# Autodesk Inventor assembly: Robot
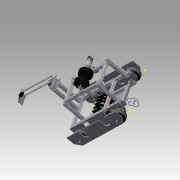
[picture p0: Inventor's stored thumbnail of the model, 180x180]
Saved by Autodesk Inventor 2016 (Build 200138000, 138)
## iProperties
Created: 2016-10-08
Part Number: Robot
Document SubType Name: Assembly
Designer: RoboticsUser
Author: RoboticsUser
## Documents named in this file (20)
- C:\Robotics\CAD\2016-17_CAD\Robot.iam
- C:\Robotics\CAD\2016-17_CAD\WheelAssemblyWFrame.iam
- C:\Robotics\CAD\COTSParts\Bosch Extrusion\Bosch 20x20 9 in.ipt
- C:\Robotics\CAD\COTSParts\Bosch Extrusion\Gusset 20x20 w screws.ipt
- C:\Robotics\CAD\COTSParts\Bosch Extrusion\Bosch 20x20 9 in - Copy.ipt
- C:\Robotics\CAD\COTSParts\Bosch Extrusion\Rexroth-6mmT-Nutm4.ipt
- C:\Robotics\CAD\COTSParts\Bosch Extrusion\Rexroth-GussetwFastenersm4x8.ipt
- C:\Robotics\CAD\COTSParts\Bosch Extrusion\Bosch 20x20 7in.ipt
- C:\Robotics\CAD\COTSParts\Bosch Extrusion\Bosch 20x20 9 in actual.ipt
- C:\Robotics\CAD\2016-17_CAD\ParticleLauncher2.0.iam
- C:\Robotics\CAD\2016-17_CAD\BBP.iam
- C:\Robotics\CAD\2016-17_CAD\ElectronicsPlate2.ipt
- C:\Robotics\CAD\COTSParts\ModernRobotics\MRI45-2204_Servo_Controller.ipt
- C:\Robotics\CAD\COTSParts\ModernRobotics\MRI45-2200_Power_Distribution_Module.ipt
- C:\Robotics\CAD\COTSParts\ModernRobotics\MRI45-2203_Motor_Controller.ipt
- C:\Robotics\CAD\COTSParts\ModernRobotics\MRI45-2201_Device_Interface.ipt
- C:\Robotics\CAD\COTSParts\Actobotics\545 parts\545400.ipt
- C:\Robotics\CAD\2016-17_CAD\PVCpipe.ipt
- C:\Robotics\CAD\COTSParts\Actobotics\545 parts\545548.ipt
- C:\Robotics\CAD\COTSParts\Actobotics\615 parts\615106.ipt
## Components (61 placed, 19 different names)
1. WheelAssemblyWFrame:1 [sub-assembly] — Mate:1, Insert:4, Insert:5, Insert:6, Flush:29, Mate:55, Flush:37, Flush:42, Mate:81, Flush:48, Flush:49, Mate:82, Flush:50, Mate:85, Flush:54, Flush:55, Mate:86
2. WheelAssemblyWFrame:2 [sub-assembly] — Mate:8, Mate:9, Flush:7, Flush:8, Insert:1, Insert:2, Insert:3, Flush:30, Flush:35, Mate:57, Mate:58, Mate:77, Mate:78, Mate:79, Flush:45, Flush:46, Flush:47, Mate:84, Flush:53, Flush:56, Mate:88, Mate:107
3. Bosch 20x20 9 in:1 — Flush:37, Mate:56, Mate:58, Mate:69, Flush:40, Mate:70, Mate:71, Mate:72, Flush:42, Mate:73, Flush:43, Mate:75, Flush:44, Mate:77
4. Gusset 20x20 w screws:1 — Mate:9, Flush:7, Mate:10, Mate:110
5. Gusset 20x20 w screws:2 — Mate:1
6. Gusset 20x20 w screws:3 — Mate:8
7. Gusset 20x20 w screws:4 — Mate:11, Flush:9
8. Bosch 20x20 9 in:2 — Mate:10, Flush:8, Mate:11, Flush:9, Flush:35, Mate:55
9. Bosch 20x20 9 in - Copy:1 — Mate:33, Flush:25, Flush:28, Flush:30, Flush:31, Mate:44, Flush:34, Mate:52, Mate:53, Mate:108, Mate:131, Mate:132, Mate:133, Mate:134, Mate:135, Flush:76
10. Rexroth-6mmT-Nutm4:1 — Insert:1
11. Rexroth-6mmT-Nutm4:2 — Insert:3, Mate:33, Flush:25
12. Rexroth-6mmT-Nutm4:3 — Insert:2
13. Bosch 20x20 9 in - Copy:2 — Mate:15, Flush:11, Mate:35, Mate:39, Flush:27, Flush:29, Flush:32, Mate:48, Flush:33, Mate:54, Mate:136, Mate:137, Mate:138, Mate:139, Flush:77
14. Rexroth-6mmT-Nutm4:4 — Insert:4
15. Rexroth-6mmT-Nutm4:5 — Insert:5
16. Rexroth-6mmT-Nutm4:6 — Insert:6, Mate:15, Flush:11
17. Bosch 20x20 9 in:3 — Flush:27, Flush:31, Mate:50, Mate:51, Mate:53, Mate:54, Flush:69
18. Bosch 20x20 9 in:4 — Mate:39, Flush:28, Flush:32, Mate:45, Mate:46, Mate:47, Mate:49, Flush:33, Flush:34, Mate:106, Mate:130
19. Gusset 20x20 w screws:5 — Mate:51, Mate:52
20. Gusset 20x20 w screws:6 — Mate:35, Mate:50
21. Gusset 20x20 w screws:7 — Mate:47, Mate:48, Mate:49
22. Gusset 20x20 w screws:8 — Mate:44, Mate:45, Mate:46
23. Rexroth-GussetwFastenersm4x8:4 — Mate:56, Mate:57
24. Gusset 20x20 w screws:11 — Mate:70, Mate:71, Mate:76
25. Gusset 20x20 w screws:12 — Mate:69, Flush:40, Mate:72, Mate:74
26. Bosch 20x20 9 in actual:1 — Mate:73, Flush:43, Mate:74, Flush:66, Mate:104, Flush:68
27. Bosch 20x20 9 in actual:2 — Mate:75, Flush:44, Mate:76, Mate:100, Mate:101, Mate:102, Flush:67, Mate:126
28. Bosch 20x20 7in:3 — Mate:79, Flush:45, Mate:80, Flush:58, Mate:91, Flush:59, Mate:94, Flush:63
29. Bosch 20x20 7in:4 — Mate:82, Mate:83, Flush:50, Mate:93, Flush:62
30. Gusset 20x20 w screws:13 — Mate:81, Flush:48, Flush:49, Mate:83
31. Gusset 20x20 w screws:14 — Mate:78, Mate:80, Flush:46, Flush:47
32. Bosch 20x20 7in:5 — Mate:84, Flush:53, Mate:89, Flush:60, Mate:98
33. Bosch 20x20 7in:6 — Mate:85, Flush:54, Mate:87, Flush:61, Mate:96, Flush:64
34. Gusset 20x20 w screws:15 — Flush:56, Mate:88, Mate:89
35. Gusset 20x20 w screws:16 — Flush:55, Mate:86, Mate:87
36. ParticleLauncher2.0:1 [sub-assembly] — Flush:58, Mate:91, Flush:59, Flush:60, Flush:61, Mate:92, Mate:95, Mate:97, Mate:99, Flush:65
37. Gusset 20x20 w screws:17 — Mate:94, Mate:95, Flush:63
38. Gusset 20x20 w screws:18 — Mate:92, Mate:93, Flush:62
39. Gusset 20x20 w screws:19 — Mate:96, Mate:97, Flush:64
40. Gusset 20x20 w screws:20 — Mate:98, Mate:99, Flush:65
41. BBP:1 [sub-assembly] — Mate:100, Mate:101, Flush:66, Mate:103, Mate:105, Mate:126
42. Gusset 20x20 w screws:21 — Mate:104, Mate:105, Flush:68
43. Gusset 20x20 w screws:22 — Mate:102, Mate:103, Flush:67
44. ElectronicsPlate2:1 — Mate:106, Flush:69, Mate:107, Mate:109, Mate:111, Mate:114, Mate:116, Mate:120, Mate:127, Mate:129
45. MRI45-2204_Servo_Controller:1 — Mate:120, Flush:73
46. MRI45-2200_Power_Distribution_Module:1 — Mate:108, Mate:109, Mate:110, Mate:112, Flush:70
47. MRI45-2203_Motor_Controller:1 — Mate:127, Flush:73, Mate:128, Flush:74
48. MRI45-2203_Motor_Controller:2 — Mate:114, Mate:115, Flush:71, Mate:117, Flush:72
49. MRI45-2203_Motor_Controller:3 — Mate:116, Mate:117, Flush:72, Mate:128, Flush:74
50. MRI45-2203_Motor_Controller:4 — Mate:111, Mate:112, Flush:70, Mate:115, Flush:71
51. MRI45-2201_Device_Interface:1 — Mate:129, Mate:130, Mate:131
52. 545400:1 — Insert:7, Insert:8
53. 545400:2 — Insert:9, Insert:10, Insert:14
54. Rexroth-6mmT-Nutm4:7 — Mate:132, Mate:133, Insert:7
55. Rexroth-6mmT-Nutm4:8 — Mate:134, Mate:135, Flush:76, Insert:8
56. Rexroth-6mmT-Nutm4:9 — Mate:136, Mate:137, Insert:10
57. Rexroth-6mmT-Nutm4:10 — Mate:138, Mate:139, Flush:77, Insert:9
58. PVCpipe:1 — Insert:12, Insert:13
59. 545548:1 — Insert:12, Insert:15
60. 545548:3 — Insert:13, Insert:14
61. 615106:1 — Insert:15
## Relationships (148: Mate 86, Flush 48, Insert 14)
- Mate:1: WheelAssemblyWFrame:1 ↔ Gusset 20x20 w screws:2
- Mate:8: WheelAssemblyWFrame:2 ↔ Gusset 20x20 w screws:3
- Mate:9: WheelAssemblyWFrame:2 ↔ Gusset 20x20 w screws:1
- Flush:7: WheelAssemblyWFrame:2 ↔ Gusset 20x20 w screws:1
- Mate:10: Gusset 20x20 w screws:1 ↔ Bosch 20x20 9 in:2
- Flush:8: WheelAssemblyWFrame:2 ↔ Bosch 20x20 9 in:2
- Mate:11: Gusset 20x20 w screws:4 ↔ Bosch 20x20 9 in:2
- Flush:9: Gusset 20x20 w screws:4 ↔ Bosch 20x20 9 in:2
- Insert:1: WheelAssemblyWFrame:2 ↔ Rexroth-6mmT-Nutm4:1
- Insert:2: WheelAssemblyWFrame:2 ↔ Rexroth-6mmT-Nutm4:3
- Insert:3: WheelAssemblyWFrame:2 ↔ Rexroth-6mmT-Nutm4:2
- Insert:4: WheelAssemblyWFrame:1 ↔ Rexroth-6mmT-Nutm4:4
- Insert:5: WheelAssemblyWFrame:1 ↔ Rexroth-6mmT-Nutm4:5
- Insert:6: WheelAssemblyWFrame:1 ↔ Rexroth-6mmT-Nutm4:6
- Mate:15: Bosch 20x20 9 in - Copy:2 ↔ Rexroth-6mmT-Nutm4:6
- Flush:11 (64.77 mm): Bosch 20x20 9 in - Copy:2 ↔ Rexroth-6mmT-Nutm4:6
- Mate:33: Bosch 20x20 9 in - Copy:1 ↔ Rexroth-6mmT-Nutm4:2
- Flush:25 (64.77 mm): Bosch 20x20 9 in - Copy:1 ↔ Rexroth-6mmT-Nutm4:2
- Mate:35: Bosch 20x20 9 in - Copy:2 ↔ Gusset 20x20 w screws:6
- Mate:39: Bosch 20x20 9 in - Copy:2 ↔ Bosch 20x20 9 in:4
- Flush:27: Bosch 20x20 9 in - Copy:2 ↔ Bosch 20x20 9 in:3
- Flush:28: Bosch 20x20 9 in - Copy:1 ↔ Bosch 20x20 9 in:4
- Flush:29 (1.6256 mm): WheelAssemblyWFrame:1 ↔ Bosch 20x20 9 in - Copy:2
- Flush:30 (1.6256 mm): WheelAssemblyWFrame:2 ↔ Bosch 20x20 9 in - Copy:1
- Flush:31 (56.896 mm): Bosch 20x20 9 in - Copy:1 ↔ Bosch 20x20 9 in:3
- Flush:32: Bosch 20x20 9 in - Copy:2 ↔ Bosch 20x20 9 in:4
- Mate:44: Bosch 20x20 9 in - Copy:1 ↔ Gusset 20x20 w screws:8
- Mate:45: Bosch 20x20 9 in:4 ↔ Gusset 20x20 w screws:8
- Mate:46: Bosch 20x20 9 in:4 ↔ Gusset 20x20 w screws:8
- Mate:47: Bosch 20x20 9 in:4 ↔ Gusset 20x20 w screws:7
- Mate:48: Bosch 20x20 9 in - Copy:2 ↔ Gusset 20x20 w screws:7
- Mate:49: Bosch 20x20 9 in:4 ↔ Gusset 20x20 w screws:7
- Flush:33: Bosch 20x20 9 in - Copy:2 ↔ Bosch 20x20 9 in:4
- Flush:34: Bosch 20x20 9 in - Copy:1 ↔ Bosch 20x20 9 in:4
- Mate:50: Bosch 20x20 9 in:3 ↔ Gusset 20x20 w screws:6
- Mate:51: Bosch 20x20 9 in:3 ↔ Gusset 20x20 w screws:5
- Mate:52: Bosch 20x20 9 in - Copy:1 ↔ Gusset 20x20 w screws:5
- Mate:53: Bosch 20x20 9 in - Copy:1 ↔ Bosch 20x20 9 in:3
- Mate:54: Bosch 20x20 9 in - Copy:2 ↔ Bosch 20x20 9 in:3
- Flush:35 (127 mm): WheelAssemblyWFrame:2 ↔ Bosch 20x20 9 in:2
- Mate:55: WheelAssemblyWFrame:1 ↔ Bosch 20x20 9 in:2
- Flush:37: WheelAssemblyWFrame:1 ↔ Bosch 20x20 9 in:1
- Mate:56: Bosch 20x20 9 in:1 ↔ Rexroth-GussetwFastenersm4x8:4
- Mate:57: WheelAssemblyWFrame:2 ↔ Rexroth-GussetwFastenersm4x8:4
- Mate:58: WheelAssemblyWFrame:2 ↔ Bosch 20x20 9 in:1
- Mate:69: Bosch 20x20 9 in:1 ↔ Gusset 20x20 w screws:12
- Flush:40: Bosch 20x20 9 in:1 ↔ Gusset 20x20 w screws:12
- Mate:70: Bosch 20x20 9 in:1 ↔ Gusset 20x20 w screws:11
- Mate:71: Bosch 20x20 9 in:1 ↔ Gusset 20x20 w screws:11
- Mate:72: Bosch 20x20 9 in:1 ↔ Gusset 20x20 w screws:12
- Flush:42: WheelAssemblyWFrame:1 ↔ Bosch 20x20 9 in:1
- Mate:73: Bosch 20x20 9 in:1 ↔ Bosch 20x20 9 in actual:1
- Flush:43: Bosch 20x20 9 in:1 ↔ Bosch 20x20 9 in actual:1
- Mate:74: Gusset 20x20 w screws:12 ↔ Bosch 20x20 9 in actual:1
- Mate:75: Bosch 20x20 9 in:1 ↔ Bosch 20x20 9 in actual:2
- Flush:44: Bosch 20x20 9 in:1 ↔ Bosch 20x20 9 in actual:2
- Mate:76: Gusset 20x20 w screws:11 ↔ Bosch 20x20 9 in actual:2
- Mate:77: WheelAssemblyWFrame:2 ↔ Bosch 20x20 9 in:1
- Mate:78: WheelAssemblyWFrame:2 ↔ Gusset 20x20 w screws:14
- Mate:79: WheelAssemblyWFrame:2 ↔ Bosch 20x20 7in:3
- Flush:45: WheelAssemblyWFrame:2 ↔ Bosch 20x20 7in:3
- Mate:80: Bosch 20x20 7in:3 ↔ Gusset 20x20 w screws:14
- Flush:46: WheelAssemblyWFrame:2 ↔ Gusset 20x20 w screws:14
- Flush:47: WheelAssemblyWFrame:2 ↔ Gusset 20x20 w screws:14
- Mate:81: WheelAssemblyWFrame:1 ↔ Gusset 20x20 w screws:13
- Flush:48: WheelAssemblyWFrame:1 ↔ Gusset 20x20 w screws:13
- Flush:49: WheelAssemblyWFrame:1 ↔ Gusset 20x20 w screws:13
- Mate:82: WheelAssemblyWFrame:1 ↔ Bosch 20x20 7in:4
- Mate:83: Bosch 20x20 7in:4 ↔ Gusset 20x20 w screws:13
- Flush:50: WheelAssemblyWFrame:1 ↔ Bosch 20x20 7in:4
- Mate:84: WheelAssemblyWFrame:2 ↔ Bosch 20x20 7in:5
- Flush:53: WheelAssemblyWFrame:2 ↔ Bosch 20x20 7in:5
- Mate:85: WheelAssemblyWFrame:1 ↔ Bosch 20x20 7in:6
- Flush:54: WheelAssemblyWFrame:1 ↔ Bosch 20x20 7in:6
- Flush:55: WheelAssemblyWFrame:1 ↔ Gusset 20x20 w screws:16
- Mate:86: WheelAssemblyWFrame:1 ↔ Gusset 20x20 w screws:16
- Mate:87: Bosch 20x20 7in:6 ↔ Gusset 20x20 w screws:16
- Flush:56: WheelAssemblyWFrame:2 ↔ Gusset 20x20 w screws:15
- Mate:88: WheelAssemblyWFrame:2 ↔ Gusset 20x20 w screws:15
- Mate:89: Bosch 20x20 7in:5 ↔ Gusset 20x20 w screws:15
- Flush:58: Bosch 20x20 7in:3 ↔ ParticleLauncher2.0:1
- Mate:91 (2.3876 mm): Bosch 20x20 7in:3 ↔ ParticleLauncher2.0:1
- Flush:59: Bosch 20x20 7in:3 ↔ ParticleLauncher2.0:1
- Flush:60: Bosch 20x20 7in:5 ↔ ParticleLauncher2.0:1
- Flush:61: Bosch 20x20 7in:6 ↔ ParticleLauncher2.0:1
- Mate:92: ParticleLauncher2.0:1 ↔ Gusset 20x20 w screws:18
- Mate:93: Bosch 20x20 7in:4 ↔ Gusset 20x20 w screws:18
- Flush:62: Bosch 20x20 7in:4 ↔ Gusset 20x20 w screws:18
- Mate:94: Bosch 20x20 7in:3 ↔ Gusset 20x20 w screws:17
- Mate:95: ParticleLauncher2.0:1 ↔ Gusset 20x20 w screws:17
- Flush:63: Bosch 20x20 7in:3 ↔ Gusset 20x20 w screws:17
- Mate:96: Bosch 20x20 7in:6 ↔ Gusset 20x20 w screws:19
- Mate:97: ParticleLauncher2.0:1 ↔ Gusset 20x20 w screws:19
- Flush:64: Bosch 20x20 7in:6 ↔ Gusset 20x20 w screws:19
- Mate:98: Bosch 20x20 7in:5 ↔ Gusset 20x20 w screws:20
- Mate:99: ParticleLauncher2.0:1 ↔ Gusset 20x20 w screws:20
- Flush:65: ParticleLauncher2.0:1 ↔ Gusset 20x20 w screws:20
- Mate:100: Bosch 20x20 9 in actual:2 ↔ BBP:1
- Mate:101: Bosch 20x20 9 in actual:2 ↔ BBP:1
- Flush:66: Bosch 20x20 9 in actual:1 ↔ BBP:1
- Mate:102: Bosch 20x20 9 in actual:2 ↔ Gusset 20x20 w screws:22
- Mate:103: BBP:1 ↔ Gusset 20x20 w screws:22
- Flush:67: Bosch 20x20 9 in actual:2 ↔ Gusset 20x20 w screws:22
- Mate:104: Bosch 20x20 9 in actual:1 ↔ Gusset 20x20 w screws:21
- Mate:105: BBP:1 ↔ Gusset 20x20 w screws:21
- Flush:68: Bosch 20x20 9 in actual:1 ↔ Gusset 20x20 w screws:21
- Mate:106: Bosch 20x20 9 in:4 ↔ ElectronicsPlate2:1
- Flush:69: Bosch 20x20 9 in:3 ↔ ElectronicsPlate2:1
- Mate:107: WheelAssemblyWFrame:2 ↔ ElectronicsPlate2:1
- Mate:108: Bosch 20x20 9 in - Copy:1 ↔ MRI45-2200_Power_Distribution_Module:1
- Mate:109: ElectronicsPlate2:1 ↔ MRI45-2200_Power_Distribution_Module:1
- Mate:110 (12.7 mm): Gusset 20x20 w screws:1 ↔ MRI45-2200_Power_Distribution_Module:1
- Mate:111: ElectronicsPlate2:1 ↔ MRI45-2203_Motor_Controller:4
- Mate:112 (20.32 mm): MRI45-2200_Power_Distribution_Module:1 ↔ MRI45-2203_Motor_Controller:4
- Flush:70: MRI45-2200_Power_Distribution_Module:1 ↔ MRI45-2203_Motor_Controller:4
- Mate:114: ElectronicsPlate2:1 ↔ MRI45-2203_Motor_Controller:2
- Mate:115 (5.08 mm): MRI45-2203_Motor_Controller:2 ↔ MRI45-2203_Motor_Controller:4
- Flush:71: MRI45-2203_Motor_Controller:2 ↔ MRI45-2203_Motor_Controller:4
- Mate:116: ElectronicsPlate2:1 ↔ MRI45-2203_Motor_Controller:3
- Mate:117 (5.08 mm): MRI45-2203_Motor_Controller:2 ↔ MRI45-2203_Motor_Controller:3
- Flush:72: MRI45-2203_Motor_Controller:2 ↔ MRI45-2203_Motor_Controller:3
- Mate:120: ElectronicsPlate2:1 ↔ MRI45-2204_Servo_Controller:1
- Mate:126: Bosch 20x20 9 in actual:2 ↔ BBP:1
- Mate:127: ElectronicsPlate2:1 ↔ MRI45-2203_Motor_Controller:1
- Flush:73: MRI45-2204_Servo_Controller:1 ↔ MRI45-2203_Motor_Controller:1
- Mate:128 (5.08 mm): MRI45-2203_Motor_Controller:1 ↔ MRI45-2203_Motor_Controller:3
- Flush:74: MRI45-2203_Motor_Controller:1 ↔ MRI45-2203_Motor_Controller:3
- Mate:129: ElectronicsPlate2:1 ↔ MRI45-2201_Device_Interface:1
- Mate:130: Bosch 20x20 9 in:4 ↔ MRI45-2201_Device_Interface:1
- Mate:131 (76.7969 mm): Bosch 20x20 9 in - Copy:1 ↔ MRI45-2201_Device_Interface:1
- Mate:132: Bosch 20x20 9 in - Copy:1 ↔ Rexroth-6mmT-Nutm4:7
- Mate:133: Bosch 20x20 9 in - Copy:1 ↔ Rexroth-6mmT-Nutm4:7
- Mate:134: Bosch 20x20 9 in - Copy:1 ↔ Rexroth-6mmT-Nutm4:8
- Mate:135: Bosch 20x20 9 in - Copy:1 ↔ Rexroth-6mmT-Nutm4:8
- Flush:76: Bosch 20x20 9 in - Copy:1 ↔ Rexroth-6mmT-Nutm4:8
- Insert:7: 545400:1 ↔ Rexroth-6mmT-Nutm4:7
- Insert:8: 545400:1 ↔ Rexroth-6mmT-Nutm4:8
- Mate:136: Bosch 20x20 9 in - Copy:2 ↔ Rexroth-6mmT-Nutm4:9
- Mate:137: Bosch 20x20 9 in - Copy:2 ↔ Rexroth-6mmT-Nutm4:9
- Mate:138: Bosch 20x20 9 in - Copy:2 ↔ Rexroth-6mmT-Nutm4:10
- Mate:139: Bosch 20x20 9 in - Copy:2 ↔ Rexroth-6mmT-Nutm4:10
- Flush:77: Bosch 20x20 9 in - Copy:2 ↔ Rexroth-6mmT-Nutm4:10
- Insert:9: 545400:2 ↔ Rexroth-6mmT-Nutm4:10
- Insert:10: 545400:2 ↔ Rexroth-6mmT-Nutm4:9
- Insert:12: PVCpipe:1 ↔ 545548:1
- Insert:13: PVCpipe:1 ↔ 545548:3
- Insert:14: 545400:2 ↔ 545548:3
- Insert:15 (4.6482 mm): 545548:1 ↔ 615106:1
